# Autodesk Inventor assembly: my1020_motor_MIR
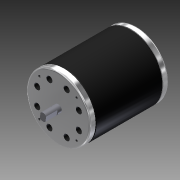
[picture p0: Inventor's stored thumbnail of the model, 180x180]
Saved by Autodesk Inventor 2012 (Build 160160000, 160)
## iProperties
Created: 2012-01-29
Part Number: my1020_motor_MIR
Document SubType Name: Assembly
Designer: Antonella Wilby
Author: Antonella Wilby
## Documents named in this file (3)
- C:\Users\Antonella\Documents\GCC Robotics 2012 - Mechanical\Robot 2.0\Drive Train\MY1020 Motor\my1020_motor_MIR.iam
- C:\Users\Antonella\Documents\GCC Robotics 2012 - Mechanical\Robot 2.0\Drive Train\MY1020 Motor\my1020_motor_MIR.ipt
- C:\Users\Antonella\Documents\GCC Robotics 2012 - Mechanical\Robot 2.0\Drive Train\MY1020 Motor\shaft_MIR.ipt
## Components (2 placed, 2 different names)
1. my1020_motor_MIR:1 — Mate:2, Mate:1
2. shaft_MIR:1 — Mate:2, Mate:1
## Relationships (2: Mate 2)
- Mate:2: my1020_motor_MIR:1 ↔ shaft_MIR:1
- Mate:1: my1020_motor_MIR:1 ↔ shaft_MIR:1
